# Autodesk Inventor assembly: TOF_golpins
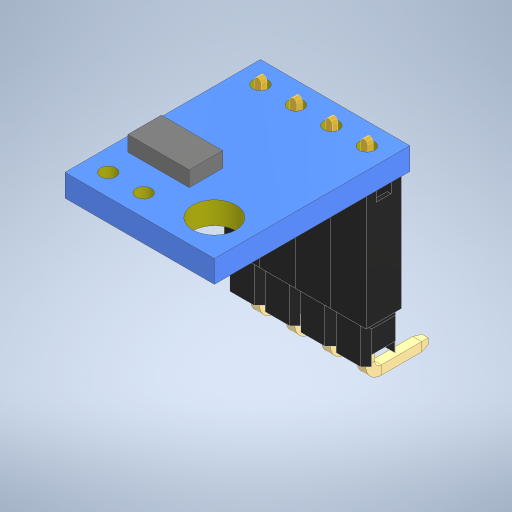
[picture p0: Inventor's stored thumbnail of the model, 512x512]
Saved by Autodesk Inventor 2023 (Build 270158000, 158)
## iProperties
Created: 2024-04-29
Part Number: TOF_golpins
Document SubType Name: Assembly
Designer: kamil
Author: kamil
## Documents named in this file (4)
- C:\Users\kamil\Documents\PROJECTS - repos\ModBot---Projekt-Zespolowy\mechanics\TOF_golpins.iam
- C:\Users\kamil\Documents\PROJECTS - repos\ModBot---Projekt-Zespolowy\mechanics\TOF_VL53L0X (1).ipt
- C:\Users\kamil\Downloads\female-header-pins-2-54-mm-pitch-1.snapshot.3\Header Pins\Header_4.ipt
- C:\Users\kamil\Downloads\1x4 Male Pin Header Angle.ipt
## Components (3 placed, 3 different names)
1. TOF_VL53L0X (1):1 — Zestawiające:1, Równoległe:1, Równoległe:2
2. Header_4:1 — Zestawiające:1, Równoległe:1, Równoległe:2, Równoległe:3, Równoległe:4, Zestawiające:2
3. 1x4 Male Pin Header Angle:1 — Równoległe:3, Równoległe:4, Zestawiające:2
## Relationships (6: Flush 4, Mate 2)
- Zestawiające:1 [Mate]: TOF_VL53L0X (1):1 ↔ Header_4:1
- Równoległe:1 [Flush] (0.3 mm): TOF_VL53L0X (1):1 ↔ Header_4:1
- Równoległe:2 [Flush] (0.3 mm): TOF_VL53L0X (1):1 ↔ Header_4:1
- Równoległe:3 [Flush]: Header_4:1 ↔ 1x4 Male Pin Header Angle:1
- Równoległe:4 [Flush]: Header_4:1 ↔ 1x4 Male Pin Header Angle:1
- Zestawiające:2 [Mate]: Header_4:1 ↔ 1x4 Male Pin Header Angle:1
